# Autodesk Inventor assembly: intake chain
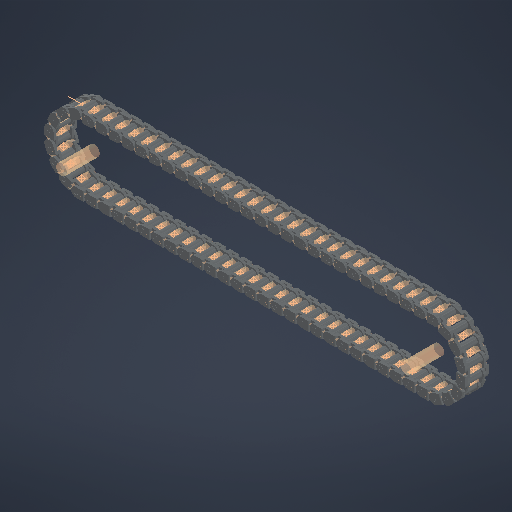
[picture p0: Inventor's stored thumbnail of the model, 512x512]
Saved by Autodesk Inventor 2025 (Build 290162000, 162)
## iProperties
RuleStatus: InUse
Created: 2020-07-07
Part Number: intake chain
Document SubType Name: Assembly
Designer: yuany
AfterDocOpen0: Open Form
Author: yuany
## Documents named in this file (3)
- C:\Users\Juan\Documents\GitHub\ATUM-VRC-High-Stakes-CAD\Protobot\intake chain.iam
- C:\Users\Juan\Documents\GitHub\ATUM-VRC-High-Stakes-CAD\VEX-CAD-Inventor\Motion\Chain Generator 6P\Workpoint Pattern.ipt
- C:\Users\Juan\Documents\GitHub\ATUM-VRC-High-Stakes-CAD\VEX-CAD-Inventor\Motion\Chain 6P\IQ Chain.ipt
## Components (69 placed, 2 different names)
1. Workpoint Pattern:1 — Mate:4, Mate:5, Angle:1
2. IQ Chain:1 — Mate:4, Mate:5, Angle:1
3. IQ Chain:2
4. IQ Chain:3
5. IQ Chain:4
6. IQ Chain:5
7. IQ Chain:6
8. IQ Chain:7
9. IQ Chain:8
10. IQ Chain:9
11. IQ Chain:10
12. IQ Chain:11
13. IQ Chain:12
14. IQ Chain:13
15. IQ Chain:14
16. IQ Chain:15
17. IQ Chain:16
18. IQ Chain:17
19. IQ Chain:18
20. IQ Chain:19
21. IQ Chain:20
22. IQ Chain:21
23. IQ Chain:22
24. IQ Chain:23
25. IQ Chain:24
26. IQ Chain:25
27. IQ Chain:26
28. IQ Chain:27
29. IQ Chain:28
30. IQ Chain:29
31. IQ Chain:30
32. IQ Chain:31
33. IQ Chain:32
34. IQ Chain:33
35. IQ Chain:34
36. IQ Chain:35
37. IQ Chain:36
38. IQ Chain:37
39. IQ Chain:38
40. IQ Chain:39
41. IQ Chain:40
42. IQ Chain:41
43. IQ Chain:42
44. IQ Chain:43
45. IQ Chain:44
46. IQ Chain:45
47. IQ Chain:46
48. IQ Chain:47
49. IQ Chain:48
50. IQ Chain:49
51. IQ Chain:50
52. IQ Chain:51
53. IQ Chain:52
54. IQ Chain:53
55. IQ Chain:54
56. IQ Chain:55
57. IQ Chain:56
58. IQ Chain:57
59. IQ Chain:58
60. IQ Chain:59
61. IQ Chain:60
62. IQ Chain:61
63. IQ Chain:62
64. IQ Chain:63
65. IQ Chain:64
66. IQ Chain:65
67. IQ Chain:66
68. IQ Chain:67
69. IQ Chain:68
## Component patterns: (68 elements, first: IQ Chain:1)
## Relationships (3: Mate 2, Angle 1)
- Mate:4: Workpoint Pattern:1 ↔ IQ Chain:1
- Mate:5: Workpoint Pattern:1 ↔ IQ Chain:1
- Angle:1 (180 deg): Workpoint Pattern:1 ↔ IQ Chain:1
## Named parameters: Center_Distance = 165.6842 mm, Sprocket1 = 32.54903 mm, Sprocket2 = 32.54903 mm, CenterDistance = 165.6842 mm
